# Autodesk Inventor assembly: joint_1_assembly
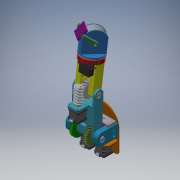
[picture p0: Inventor's stored thumbnail of the model, 180x180]
Saved by Autodesk Inventor 2019 (Build 230136000, 136)
## iProperties
Created: 2019-12-25
Part Number: joint_1_assembly
Material: Типовые
Document SubType Name: Assembly
Designer: Петров Иван
Author: Петров Иван
## Documents named in this file (21)
- E:\IVAN\Ivan_desktop\GitHub\Arm_manip\hardware\joint_1_assembly.iam
- E:\IVAN\Ivan_desktop\GitHub\Arm_manip\hardware\joint_1_base.ipt
- E:\IVAN\Ivan_desktop\GitHub\Arm_manip\hardware\Standart_things\Nema 17HS4401-S.ipt
- E:\IVAN\Ivan_desktop\GitHub\Arm_manip\hardware\Standart_things\Подшипник 17x23x4.ipt
- E:\IVAN\Ivan_desktop\GitHub\Arm_manip\hardware\joint_1_stand.ipt
- E:\IVAN\Ivan_desktop\GitHub\Arm_manip\hardware\joint1_gear.ipt
- E:\IVAN\Ivan_desktop\GitHub\Arm_manip\hardware\joint_1_assembly\Мастер проектирования\Червячная передача1.iam
- E:\IVAN\Ivan_desktop\GitHub\Arm_manip\hardware\joint_1_assembly\Мастер проектирования\Червячная передача3.iam
- E:\IVAN\Ivan_desktop\GitHub\Arm_manip\hardware\joint1_gear_holder.ipt
- E:\IVAN\Ivan_desktop\GitHub\Arm_manip\hardware\Standart_things\Подшипник 4x8x3.ipt
- E:\IVAN\Ivan_desktop\GitHub\Arm_manip\hardware\joint1_level.ipt
- E:\IVAN\Ivan_desktop\GitHub\Arm_manip\hardware\joint1_level_part_2.ipt
- E:\IVAN\Ivan_desktop\GitHub\Arm_manip\hardware\joint_1_assembly\Мастер проектирования\Червячная передача5.iam
- E:\IVAN\Ivan_desktop\GitHub\Arm_manip\hardware\joint_1_os.ipt
- E:\IVAN\Ivan_desktop\GitHub\Arm_manip\hardware\joint_2_part1.ipt
- E:\IVAN\Ivan_desktop\GitHub\Arm_manip\hardware\Standart_things\tower prone.ipt
- E:\IVAN\Ivan_desktop\GitHub\Arm_manip\hardware\joint2_rotate_mec.ipt
- E:\IVAN\Ivan_desktop\GitHub\Arm_manip\hardware\joint_1_assembly\Мастер проектирования\Цилиндрическое зубчатое зацепление3.iam
- E:\IVAN\Ivan_desktop\GitHub\Arm_manip\hardware\Standart_things\Potentiometer.ipt
- E:\IVAN\Ivan_desktop\GitHub\Arm_manip\hardware\joint2_rotate_mec_patr2.ipt
- E:\IVAN\Ivan_desktop\GitHub\Arm_manip\hardware\joint3_as.iam
## Components (30 placed, 18 different names)
1. joint_1_base:1 — Совмещение:1, Совмещение:2, Совмещение:3, Совмещение:4, Совмещение:5, Совмещение:6, Заподлицо:1, Совмещение:7, Заподлицо:2, Совмещение:8, Совмещение:10, Совмещение:11, Заподлицо:3, Совмещение:12, Совмещение:13, Заподлицо:4, Угол:1, Угол:3
2. Nema 17HS4401-S:1 — Совмещение:1, Совмещение:2, Совмещение:3, Совмещение:33
3. Nema 17HS4401-S:2 — Совмещение:4, Совмещение:5, Совмещение:6, Совмещение:31
4. Подшипник 17x23x4:1 — Заподлицо:1, Совмещение:7
5. Подшипник 17x23x4:2 — Заподлицо:2, Совмещение:8
6. joint_1_stand:1 — Совмещение:10, Совмещение:11, Заподлицо:3, Заподлицо:5, Совмещение:14, Совмещение:36
7. joint_1_stand:2 — Совмещение:12, Совмещение:13, Заподлицо:4, Совмещение:16, Заподлицо:6, Совмещение:27, Заподлицо:7, Угол:2, Угол:8
8. Подшипник 17x23x4:3 — Совмещение:16, Заподлицо:6
9. Подшипник 17x23x4:4 — Заподлицо:5, Совмещение:14
10. joint1_gear:1 — Совмещение:27, Заподлицо:7, Совмещение:32, Совмещение:34, Совмещение:42, Совмещение:43, Совмещение:85, Совмещение:86
11. Червячная передача:1 [sub-assembly] — Совмещение:31, Угол:1, Совмещение:32, Угол:2, Совмещение:39, Совмещение:44, Совмещение:85
12. Червячная передача:2 [sub-assembly] — Совмещение:33, Угол:3, Совмещение:34, Совмещение:38, Совмещение:86
13. joint1_gear_holder:1 — Совмещение:36, Совмещение:38, Совмещение:39, Совмещение:40, Заподлицо:8, Совмещение:41, Заподлицо:9
14. Подшипник 4x8x3:1 — Совмещение:40, Заподлицо:8
15. Подшипник 4x8x3:2 — Совмещение:41, Заподлицо:9
16. joint1_level:1 — Совмещение:42, Совмещение:43, Совмещение:44, Совмещение:45, Совмещение:46, Совмещение:47, Угол:8
17. joint1_level_part_2:1 — Совмещение:45, Совмещение:46, Совмещение:47, Совмещение:48, Угол:5, Угол:6, Совмещение:51, Заподлицо:11, Совмещение:52, Заподлицо:12, Заподлицо:13, Совмещение:56, Совмещение:57, Совмещение:58, Совмещение:60, Совмещение:63, Угол:7
18. Nema 17HS4401-S:3 — Совмещение:48, Совмещение:50, Совмещение:56, Совмещение:57, Совмещение:58, Совмещение:59
19. Червячная передача:3 [sub-assembly] — Совмещение:50, Угол:5, Угол:6, Совмещение:54, Совмещение:55
20. Подшипник 17x23x4:5 — Совмещение:52, Заподлицо:12
21. Подшипник 17x23x4:6 — Совмещение:51, Заподлицо:11, Совмещение:53
22. joint_1_os:1 — Совмещение:53, Заподлицо:13, Совмещение:54, Совмещение:55, Совмещение:61, Совмещение:62
23. Подшипник 17x23x4:7 — Совмещение:59, Совмещение:60
24. joint_2_part1:1 — Совмещение:61, Совмещение:62, Совмещение:63, Совмещение:64, Совмещение:65, Совмещение:66, Угол:7
25. joint2_rotate_mec:1 — Совмещение:64, Совмещение:65, Совмещение:66, Совмещение:67, Совмещение:68, Совмещение:69, Совмещение:74, Совмещение:75, Совмещение:76, Совмещение:77, Совмещение:78, Совмещение:80, Совмещение:83, Совмещение:87
26. tower prone:4 — Совмещение:67, Совмещение:68, Совмещение:69, Совмещение:79
27. Цилиндрическое зубчатое зацепление:1 [sub-assembly] — Совмещение:77, Совмещение:78, Совмещение:79, Совмещение:80
28. Potentiometer:1 — Совмещение:74, Совмещение:75, Совмещение:76
29. joint2_rotate_mec_patr2:1 — Совмещение:83, Совмещение:87, Совмещение:88, Совмещение:89, Совмещение:90
30. joint3_as:1 [sub-assembly] — Совмещение:88, Совмещение:89, Совмещение:90
## Relationships (84: Mate 65, Flush 12, Angle 7)
- Совмещение:1 [Mate]: joint_1_base:1 ↔ Nema 17HS4401-S:1
- Совмещение:2 [Mate]: joint_1_base:1 ↔ Nema 17HS4401-S:1
- Совмещение:3 [Mate]: joint_1_base:1 ↔ Nema 17HS4401-S:1
- Совмещение:4 [Mate]: joint_1_base:1 ↔ Nema 17HS4401-S:2
- Совмещение:5 [Mate]: joint_1_base:1 ↔ Nema 17HS4401-S:2
- Совмещение:6 [Mate]: joint_1_base:1 ↔ Nema 17HS4401-S:2
- Заподлицо:1 [Flush]: joint_1_base:1 ↔ Подшипник 17x23x4:1
- Совмещение:7 [Mate]: joint_1_base:1 ↔ Подшипник 17x23x4:1
- Заподлицо:2 [Flush]: joint_1_base:1 ↔ Подшипник 17x23x4:2
- Совмещение:8 [Mate]: joint_1_base:1 ↔ Подшипник 17x23x4:2
- Совмещение:10 [Mate] (10 mm): joint_1_base:1 ↔ joint_1_stand:1
- Совмещение:11 [Mate]: joint_1_base:1 ↔ joint_1_stand:1
- Заподлицо:3 [Flush]: joint_1_base:1 ↔ joint_1_stand:1
- Совмещение:12 [Mate]: joint_1_base:1 ↔ joint_1_stand:2
- Совмещение:13 [Mate] (10 mm): joint_1_base:1 ↔ joint_1_stand:2
- Заподлицо:4 [Flush]: joint_1_base:1 ↔ joint_1_stand:2
- Заподлицо:5 [Flush]: joint_1_stand:1 ↔ Подшипник 17x23x4:4
- Совмещение:14 [Mate]: joint_1_stand:1 ↔ Подшипник 17x23x4:4
- Совмещение:16 [Mate]: joint_1_stand:2 ↔ Подшипник 17x23x4:3
- Заподлицо:6 [Flush]: joint_1_stand:2 ↔ Подшипник 17x23x4:3
- Совмещение:27 [Mate]: joint_1_stand:2 ↔ joint1_gear:1
- Заподлицо:7 [Flush]: joint_1_stand:2 ↔ joint1_gear:1
- Совмещение:31 [Mate]: Nema 17HS4401-S:2 ↔ Червячная передача:1
- Угол:1 [Angle] (0 deg): joint_1_base:1 ↔ Червячная передача:1
- Совмещение:32 [Mate]: joint1_gear:1 ↔ Червячная передача:1
- Угол:2 [Angle] (0 deg): joint_1_stand:2 ↔ Червячная передача:1
- Совмещение:33 [Mate]: Nema 17HS4401-S:1 ↔ Червячная передача:2
- Угол:3 [Angle] (0 deg): joint_1_base:1 ↔ Червячная передача:2
- Совмещение:34 [Mate]: joint1_gear:1 ↔ Червячная передача:2
- Совмещение:36 [Mate]: joint_1_stand:1 ↔ joint1_gear_holder:1
- Совмещение:38 [Mate]: Червячная передача:2 ↔ joint1_gear_holder:1
- Совмещение:39 [Mate]: Червячная передача:1 ↔ joint1_gear_holder:1
- Совмещение:40 [Mate]: joint1_gear_holder:1 ↔ Подшипник 4x8x3:1
- Заподлицо:8 [Flush]: joint1_gear_holder:1 ↔ Подшипник 4x8x3:1
- Совмещение:41 [Mate]: joint1_gear_holder:1 ↔ Подшипник 4x8x3:2
- Заподлицо:9 [Flush]: joint1_gear_holder:1 ↔ Подшипник 4x8x3:2
- Совмещение:42 [Mate]: joint1_gear:1 ↔ joint1_level:1
- Совмещение:43 [Mate]: joint1_gear:1 ↔ joint1_level:1
- Совмещение:44 [Mate]: Червячная передача:1 ↔ joint1_level:1
- Совмещение:45 [Mate]: joint1_level:1 ↔ joint1_level_part_2:1
- Совмещение:46 [Mate]: joint1_level:1 ↔ joint1_level_part_2:1
- Совмещение:47 [Mate]: joint1_level:1 ↔ joint1_level_part_2:1
- Совмещение:48 [Mate]: joint1_level_part_2:1 ↔ Nema 17HS4401-S:3
- Совмещение:50 [Mate]: Nema 17HS4401-S:3 ↔ Червячная передача:3
- Угол:5 [Angle] (0 deg): joint1_level_part_2:1 ↔ Червячная передача:3
- Угол:6 [Angle] (0 deg): joint1_level_part_2:1 ↔ Червячная передача:3
- Совмещение:51 [Mate]: joint1_level_part_2:1 ↔ Подшипник 17x23x4:6
- Заподлицо:11 [Flush]: joint1_level_part_2:1 ↔ Подшипник 17x23x4:6
- Совмещение:52 [Mate]: joint1_level_part_2:1 ↔ Подшипник 17x23x4:5
- Заподлицо:12 [Flush]: joint1_level_part_2:1 ↔ Подшипник 17x23x4:5
- Совмещение:53 [Mate]: Подшипник 17x23x4:6 ↔ joint_1_os:1
- Заподлицо:13 [Flush]: joint1_level_part_2:1 ↔ joint_1_os:1
- Совмещение:54 [Mate]: Червячная передача:3 ↔ joint_1_os:1
- Совмещение:55 [Mate]: Червячная передача:3 ↔ joint_1_os:1
- Совмещение:56 [Mate]: joint1_level_part_2:1 ↔ Nema 17HS4401-S:3
- Совмещение:57 [Mate]: joint1_level_part_2:1 ↔ Nema 17HS4401-S:3
- Совмещение:58 [Mate]: joint1_level_part_2:1 ↔ Nema 17HS4401-S:3
- Совмещение:59 [Mate]: Nema 17HS4401-S:3 ↔ Подшипник 17x23x4:7
- Совмещение:60 [Mate]: joint1_level_part_2:1 ↔ Подшипник 17x23x4:7
- Совмещение:61 [Mate]: joint_1_os:1 ↔ joint_2_part1:1
- Совмещение:62 [Mate]: joint_1_os:1 ↔ joint_2_part1:1
- Совмещение:63 [Mate] (0.4 mm): joint1_level_part_2:1 ↔ joint_2_part1:1
- Совмещение:64 [Mate]: joint_2_part1:1 ↔ joint2_rotate_mec:1
- Совмещение:65 [Mate]: joint_2_part1:1 ↔ joint2_rotate_mec:1
- Совмещение:66 [Mate]: joint_2_part1:1 ↔ joint2_rotate_mec:1
- Совмещение:67 [Mate]: joint2_rotate_mec:1 ↔ tower prone:4
- Совмещение:68 [Mate]: joint2_rotate_mec:1 ↔ tower prone:4
- Совмещение:69 [Mate]: joint2_rotate_mec:1 ↔ tower prone:4
- Совмещение:74 [Mate]: joint2_rotate_mec:1 ↔ Potentiometer:1
- Совмещение:75 [Mate]: joint2_rotate_mec:1 ↔ Potentiometer:1
- Совмещение:76 [Mate]: joint2_rotate_mec:1 ↔ Potentiometer:1
- Совмещение:77 [Mate]: joint2_rotate_mec:1 ↔ Цилиндрическое зубчатое зацепление:1
- Совмещение:78 [Mate]: joint2_rotate_mec:1 ↔ Цилиндрическое зубчатое зацепление:1
- Совмещение:79 [Mate]: tower prone:4 ↔ Цилиндрическое зубчатое зацепление:1
- Совмещение:80 [Mate]: joint2_rotate_mec:1 ↔ Цилиндрическое зубчатое зацепление:1
- Совмещение:83 [Mate]: joint2_rotate_mec:1 ↔ joint2_rotate_mec_patr2:1
- Совмещение:85 [Mate]: joint1_gear:1 ↔ Червячная передача:1
- Совмещение:86 [Mate]: joint1_gear:1 ↔ Червячная передача:2
- Угол:7 [Angle] (0 deg): joint1_level_part_2:1 ↔ joint_2_part1:1
- Угол:8 [Angle] (0 deg): joint_1_stand:2 ↔ joint1_level:1
- Совмещение:87 [Mate]: joint2_rotate_mec:1 ↔ joint2_rotate_mec_patr2:1
- Совмещение:88 [Mate]: joint2_rotate_mec_patr2:1 ↔ joint3_as:1
- Совмещение:89 [Mate]: joint2_rotate_mec_patr2:1 ↔ joint3_as:1
- Совмещение:90 [Mate]: joint2_rotate_mec_patr2:1 ↔ joint3_as:1
